# Autodesk Inventor assembly: idler_screw_join_mirrored
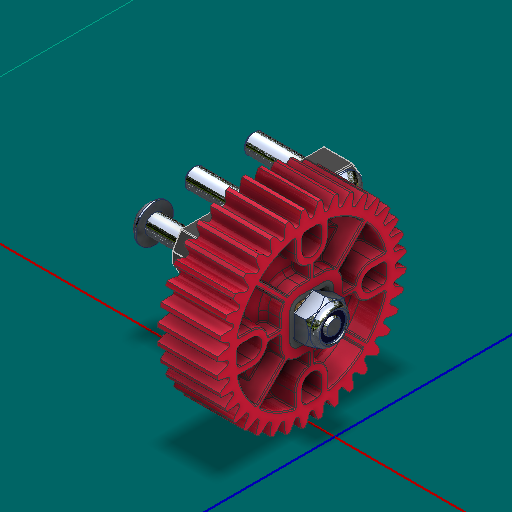
[picture p0: Inventor's stored thumbnail of the model, 512x512]
Saved by Autodesk Inventor 2025 (Build 290162000, 162)
## iProperties
Created: 2024-08-16
Part Number: idler_screw_join_mirrored
Document SubType Name: Assembly
Designer: averey
Author: averey
## Documents named in this file (9)
- C:\Users\avere\vex_robotics_high_stakes\hardware\cad\ATLAS\chassis\drive_pod\back_left\gearbox\idler_screw_join_mirrored.iam
- C:\Users\avere\vex_robotics_high_stakes\hardware\cad\ATLAS\chassis\drive_pod\back_left\gearbox\Bearing Flat Low Profile_mirrored.ipt
- C:\Users\avere\vex_robotics_high_stakes\hardware\cad\ATLAS\chassis\drive_pod\back_left\gearbox\Nut Thin Nylock_mirrored.ipt
- C:\Users\avere\vex_robotics_high_stakes\hardware\cad\VEX-CAD-Inventor\Motion\Spacers\Washer Steel\SWasher .375 OD x .062500.ipt
- C:\Users\avere\vex_robotics_high_stakes\hardware\cad\VEX-CAD-Inventor\Motion\Spacers\Washer Steel.ipt
- C:\Users\avere\vex_robotics_high_stakes\hardware\cad\ATLAS\chassis\drive_pod\back_left\gearbox\HS 36T Gear, Circle_mirrored.iam
- C:\Users\avere\vex_robotics_high_stakes\hardware\cad\VEX-CAD-Inventor\Structure\Hardware\Screw Steel - Star\SScrew Star Smooth .750.ipt
- C:\Users\avere\vex_robotics_high_stakes\hardware\cad\VEX-CAD-Inventor\Structure\Hardware\Screw Steel - Star.ipt
- C:\Users\avere\vex_robotics_high_stakes\hardware\cad\VEX-CAD-Inventor\Structure\Hardware\Screw Steel - Star\SScrew Star Smooth 1.500.ipt
## Components (8 placed, 6 different names)
1. Bearing Flat Low Profile_mirrored:1 — Angle:1, Insert:2, Insert:7, Insert:6, Insert:8
2. Nut Thin Nylock_mirrored:1 — Insert:2, Insert:3
3. SWasher .375 OD x .062500:1 — Insert:3, Insert:4
4. Nut Thin Nylock_mirrored:2 — Insert:5
5. HS 36T Gear, Circle_mirrored:1 [sub-assembly] — Insert:5, Insert:4
6. SScrew Star Smooth .750:1 — Insert:7
7. SScrew Star Smooth .750:2 — Insert:6
8. SScrew Star Smooth 1.500:3 — Insert:8
## Relationships (8: Insert 7, Angle 1)
- Angle:1 (0 deg): Bearing Flat Low Profile_mirrored:1
- Insert:2 (1.27 mm): Bearing Flat Low Profile_mirrored:1 ↔ Nut Thin Nylock_mirrored:1
- Insert:3: Nut Thin Nylock_mirrored:1 ↔ SWasher .375 OD x .062500:1
- Insert:5: Nut Thin Nylock_mirrored:2 ↔ HS 36T Gear, Circle_mirrored:1
- Insert:4: SWasher .375 OD x .062500:1 ↔ HS 36T Gear, Circle_mirrored:1
- Insert:7 (1.27 mm): Bearing Flat Low Profile_mirrored:1 ↔ SScrew Star Smooth .750:1
- Insert:6 (1.27 mm): Bearing Flat Low Profile_mirrored:1 ↔ SScrew Star Smooth .750:2
- Insert:8 (7.9375 mm): Bearing Flat Low Profile_mirrored:1 ↔ SScrew Star Smooth 1.500:3
